# Autodesk Inventor assembly: Inner Channel
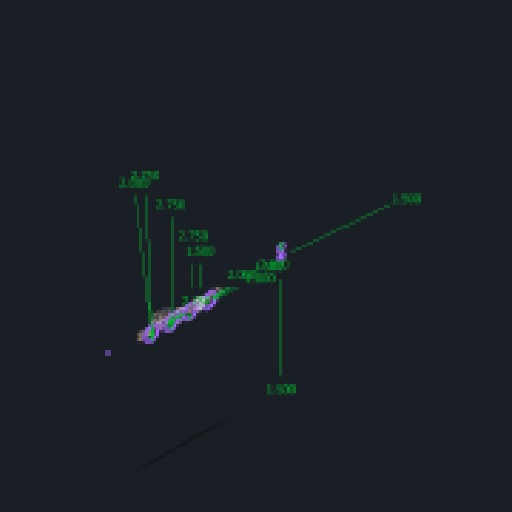
[picture p0: Inventor's stored thumbnail of the model, 512x512]
Saved by Autodesk Inventor 2025.1 (Build 291241000, 241)
## iProperties
Created: 2024-11-04
Part Number: Inner Channel
Document SubType Name: Assembly
Designer: avere
Author: avere
## Documents named in this file (28)
- C:\Users\avere\VEX\High Stakes\CAD\V3\Chassis\Drivebay Right\Inner Channel.iam
- C:\Users\avere\VEX\High Stakes\CAD\V3\Chassis\Drivebay Right\Alu C 1x2x1x30.ipt
- C:\Users\avere\VEX\High Stakes\CAD\V3\Chassis\Drivebay Right\Alu C 1x2x1x6.ipt
- C:\Users\avere\VEX\High Stakes\CAD\V3\Chassis\Drivebay Right\Bearing Flat.ipt
- C:\Users\avere\VEX\High Stakes\CAD\ROBOPROS-CAD-Inventor\Motion\Spacers\Spacer Nylon .500 OD\NSpacer White .500 OD x .250.ipt
- C:\Users\avere\VEX\High Stakes\CAD\ROBOPROS-CAD-Inventor\Motion\Spacers\Spacer Nylon .500 OD.ipt
- C:\Users\avere\VEX\High Stakes\CAD\V3\Chassis\Drivebay Right\Bearing Flat NScrew Slotted Offset.iam
- C:\Users\avere\VEX\High Stakes\CAD\ROBOPROS-CAD-Inventor\Structure\Hardware\Screw Steel - Star\SScrew Star Smooth 1.750.ipt
- C:\Users\avere\VEX\High Stakes\CAD\ROBOPROS-CAD-Inventor\Structure\Hardware\Screw Steel - Star.ipt
- C:\Users\avere\VEX\High Stakes\CAD\ROBOPROS-CAD-Inventor\Structure\Hardware\Screw Steel - Star\SScrew Star Smooth .250.ipt
- C:\Users\avere\VEX\High Stakes\CAD\V3\Chassis\Drivebay Right\Nylon Standoff .875.ipt
- C:\Users\avere\VEX\High Stakes\CAD\ROBOPROS-CAD-Inventor\Motion\Spacers\Spacer Nylon .375 OD\NSpacer .375 OD x .500.ipt
- C:\Users\avere\VEX\High Stakes\CAD\ROBOPROS-CAD-Inventor\Motion\Spacers\Spacer Nylon .375 OD.ipt
- C:\Users\avere\VEX\High Stakes\CAD\ROBOPROS-CAD-Inventor\Structure\Hardware\Nut Nylon\Nut Nylon - White.ipt
- C:\Users\avere\VEX\High Stakes\CAD\ROBOPROS-CAD-Inventor\Structure\Hardware\Nut Nylon.ipt
- C:\Users\avere\VEX\High Stakes\CAD\ROBOPROS-CAD-Inventor\Structure\Hardware\Screw Shoulder Robosource\SScrew Shoulder Smooth 2.000 x .04.ipt
- C:\Users\avere\VEX\High Stakes\CAD\ROBOPROS-CAD-Inventor\Structure\Hardware\Screw Shoulder Robosource.ipt
- C:\Users\avere\VEX\High Stakes\CAD\V3\Chassis\Drivebay Right\Bearing Flat Low Profile 2-Hole.ipt
- C:\Users\avere\VEX\High Stakes\CAD\V3\Chassis\Drivebay Right\1-Post Hex Nut Retainer With Nylon Hardware.iam
- C:\Users\avere\VEX\High Stakes\CAD\V3\Chassis\Drivebay Right\Bearing Flat NScrew Slotted.iam
- C:\Users\avere\VEX\High Stakes\CAD\V3\Chassis\Drivebay Right\Nut Nylon Thread-Forming.ipt
- C:\Users\avere\VEX\High Stakes\CAD\V3\Chassis\Drivebay Right\NScrew Slotted Threaded .500.ipt
- C:\Users\avere\VEX\High Stakes\CAD\V3\Chassis\Drivebay Right\NScrew Pan Head Threaded .250.ipt
- C:\Users\avere\VEX\High Stakes\CAD\ROBOPROS-CAD-Inventor\Structure\Hardware\Screw Shoulder Robosource\SScrew Shoulder Smooth .375 x .12.ipt
- C:\Users\avere\VEX\High Stakes\CAD\ROBOPROS-CAD-Inventor\Motion\Spacers\Spacer Nylon .500 OD\NSpacer White .500 OD x .125.ipt
- C:\Users\avere\VEX\High Stakes\CAD\ROBOPROS-CAD-Inventor\Motion\Spacers\Washer Steel\SWasher .500 OD x .062500\SWasher .500 OD x .062500.ipt
- C:\Users\avere\VEX\High Stakes\CAD\ROBOPROS-CAD-Inventor\Motion\Spacers\Washer Steel\SWasher .500 OD x .062500.ipt
- C:\Users\avere\VEX\High Stakes\CAD\ROBOPROS-CAD-Inventor\Motion\Shaft LS\Bearing Flat.ipt
## Components (56 placed, 20 different names)
1. Alu C 1x2x1x30:1 — Flush:2, Flush:3, Flush:1, Mate:19, Insert:58, Mate:21, Insert:62, Insert:63, Insert:61, Insert:45, Insert:44, Insert:46, Insert:47, Mate:15, Insert:50, Insert:55, Mate:17, Insert:56, Insert:67, Insert:68, Insert:69, Insert:76, Insert:77, Insert:75, Mate:25, Insert:74, Insert:79, Insert:80, Insert:78, Mate:28, Insert:84, Mate:29, Insert:85, Insert:86, Insert:89, Insert:88, Insert:94, Insert:95, Insert:54, Mate:13, Insert:55, Insert:56, Insert:57, Mate:14
2. Alu C 1x2x1x6:1 — Insert:64, Insert:32, Insert:39, Insert:81, Insert:82, Insert:92, Insert:91, Insert:93, Insert:96, Insert:97, Insert:100
3. Bearing Flat:1 — Mate:21, Insert:62, Insert:99
4. Bearing Flat:2 — Insert:63, Insert:20
5. NSpacer White .500 OD x .250:1 — Insert:64, Insert:20
6. SScrew Star Smooth 1.750:1 — Insert:61
7. SScrew Star Smooth .250:2 — Insert:32
8. Nylon Standoff .875:1 — Insert:39
9. NSpacer .375 OD x .500:1 — Insert:54, Insert:51
10. NSpacer .375 OD x .500:2 — Insert:53, Insert:52
11. Nut Nylon - White:1 — Insert:45
12. Nut Nylon - White:2 — Insert:44
13. Nut Nylon - White:3 — Insert:46
14. Nut Nylon - White:4 — Insert:47
15. SScrew Shoulder Smooth 2.000 x .04:1 — Insert:53, Mate:16
16. SScrew Shoulder Smooth 2.000 x .04:2 — Insert:54
17. Bearing Flat Low Profile 2-Hole:1 — Insert:52, Insert:51, Mate:15, Insert:50
18. 1-Post Hex Nut Retainer With Nylon Hardware:1 [sub-assembly] — Mate:16, Insert:55
19. 1-Post Hex Nut Retainer With Nylon Hardware:2 [sub-assembly] — Mate:17, Insert:56
20. NSpacer .375 OD x .500:3 — Insert:73, Insert:70
21. NSpacer .375 OD x .500:4 — Insert:72, Insert:71
22. Nut Nylon - White:5 — Insert:76
23. Nut Nylon - White:6 — Insert:77
24. Nut Nylon - White:7 — Insert:75
25. SScrew Shoulder Smooth 2.000 x .04:3 — Insert:72, Mate:24
26. SScrew Shoulder Smooth 2.000 x .04:4 — Insert:73, Mate:26
27. Bearing Flat Low Profile 2-Hole:2 — Mate:25, Insert:74, Insert:71, Insert:70
28. 1-Post Hex Nut Retainer With Nylon Hardware:3 [sub-assembly] — Insert:79, Mate:24
29. 1-Post Hex Nut Retainer With Nylon Hardware:4 [sub-assembly] — Mate:26, Insert:80
30. Nut Nylon - White:8 — Insert:78
31. Bearing Flat NScrew Slotted:1 [sub-assembly] — Mate:19, Insert:58
32. Nylon Standoff .875:2 — Insert:67
33. Nylon Standoff .875:3 — Insert:68
34. Nylon Standoff .875:4 — Insert:69
35. Nut Nylon Thread-Forming:1 — Insert:81
36. Nut Nylon Thread-Forming:2 — Insert:82
37. Bearing Flat NScrew Slotted Offset:2 [sub-assembly] — Mate:28, Insert:84
38. Bearing Flat Low Profile 2-Hole:3 — Mate:29, Insert:85, Insert:87
39. NScrew Slotted Threaded .500:1 — Insert:86
40. Nut Nylon - White:9 — Insert:87
41. Nut Nylon - White:10 — Insert:89
42. Nut Nylon - White:11 — Insert:88
43. NScrew Pan Head Threaded .250:1 — Insert:92
44. NScrew Pan Head Threaded .250:2 — Insert:91
45. Nylon Standoff .875:5 — Insert:94
46. SScrew Star Smooth .250:3 — Insert:95
47. SScrew Star Smooth 1.750:4 — Insert:93
48. SScrew Shoulder Smooth .375 x .12:5 — Insert:96
49. Nut Nylon Thread-Forming:3 — Insert:97
50. NSpacer White .500 OD x .125:2 — Insert:99, Insert:98
51. SWasher .500 OD x .062500:1 — Insert:100, Insert:98
52. Bearing Flat Low Profile 2-Hole:4 — Insert:54
53. NScrew Slotted Threaded .500:2 — Insert:55
54. Nut Nylon - White:12 — Mate:13
55. Nylon Standoff .875:6 — Insert:56
56. Bearing Flat:3 — Insert:57, Mate:14
## Relationships (71: Insert 56, Mate 13, Flush 2)
- Flush:2 (-38.1 mm): Alu C 1x2x1x30:1
- Flush:3 (-7.9375 mm): Alu C 1x2x1x30:1
- Flush:1 [Mate] (-190.5 mm): Alu C 1x2x1x30:1
- Mate:19: Alu C 1x2x1x30:1 ↔ Bearing Flat NScrew Slotted:1
- Insert:58: Alu C 1x2x1x30:1 ↔ Bearing Flat NScrew Slotted:1
- Mate:21: Alu C 1x2x1x30:1 ↔ Bearing Flat:1
- Insert:62: Alu C 1x2x1x30:1 ↔ Bearing Flat:1
- Insert:63: Alu C 1x2x1x30:1 ↔ Bearing Flat:2
- Insert:64: Alu C 1x2x1x6:1 ↔ NSpacer White .500 OD x .250:1
- Insert:20: Bearing Flat:2 ↔ NSpacer White .500 OD x .250:1
- Insert:61: Alu C 1x2x1x30:1 ↔ SScrew Star Smooth 1.750:1
- Insert:32: Alu C 1x2x1x6:1 ↔ SScrew Star Smooth .250:2
- Insert:39: Alu C 1x2x1x6:1 ↔ Nylon Standoff .875:1
- Insert:45: Alu C 1x2x1x30:1 ↔ Nut Nylon - White:1
- Insert:44: Alu C 1x2x1x30:1 ↔ Nut Nylon - White:2
- Insert:46: Alu C 1x2x1x30:1 ↔ Nut Nylon - White:3
- Insert:47: Alu C 1x2x1x30:1 ↔ Nut Nylon - White:4
- Insert:53 (1.5875 mm): NSpacer .375 OD x .500:2 ↔ SScrew Shoulder Smooth 2.000 x .04:1
- Insert:54 (1.5875 mm): NSpacer .375 OD x .500:1 ↔ SScrew Shoulder Smooth 2.000 x .04:2
- Insert:52 (1.27 mm): NSpacer .375 OD x .500:2 ↔ Bearing Flat Low Profile 2-Hole:1
- Insert:51 (1.27 mm): NSpacer .375 OD x .500:1 ↔ Bearing Flat Low Profile 2-Hole:1
- Mate:15: Alu C 1x2x1x30:1 ↔ Bearing Flat Low Profile 2-Hole:1
- Insert:50: Alu C 1x2x1x30:1 ↔ Bearing Flat Low Profile 2-Hole:1
- Mate:16: SScrew Shoulder Smooth 2.000 x .04:1 ↔ 1-Post Hex Nut Retainer With Nylon Hardware:1
- Insert:55: Alu C 1x2x1x30:1 ↔ 1-Post Hex Nut Retainer With Nylon Hardware:1
- Mate:17: Alu C 1x2x1x30:1 ↔ 1-Post Hex Nut Retainer With Nylon Hardware:2
- Insert:56: Alu C 1x2x1x30:1 ↔ 1-Post Hex Nut Retainer With Nylon Hardware:2
- Insert:67: Alu C 1x2x1x30:1 ↔ Nylon Standoff .875:2
- Insert:68: Alu C 1x2x1x30:1 ↔ Nylon Standoff .875:3
- Insert:69: Alu C 1x2x1x30:1 ↔ Nylon Standoff .875:4
- Insert:76: Alu C 1x2x1x30:1 ↔ Nut Nylon - White:5
- Insert:77: Alu C 1x2x1x30:1 ↔ Nut Nylon - White:6
- Insert:75: Alu C 1x2x1x30:1 ↔ Nut Nylon - White:7
- Insert:72 (1.5875 mm): NSpacer .375 OD x .500:4 ↔ SScrew Shoulder Smooth 2.000 x .04:3
- Insert:73 (1.5875 mm): NSpacer .375 OD x .500:3 ↔ SScrew Shoulder Smooth 2.000 x .04:4
- Mate:25: Alu C 1x2x1x30:1 ↔ Bearing Flat Low Profile 2-Hole:2
- Insert:74: Alu C 1x2x1x30:1 ↔ Bearing Flat Low Profile 2-Hole:2
- Insert:71 (1.27 mm): NSpacer .375 OD x .500:4 ↔ Bearing Flat Low Profile 2-Hole:2
- Insert:70 (1.27 mm): NSpacer .375 OD x .500:3 ↔ Bearing Flat Low Profile 2-Hole:2
- Insert:79: Alu C 1x2x1x30:1 ↔ 1-Post Hex Nut Retainer With Nylon Hardware:3
- Mate:24: SScrew Shoulder Smooth 2.000 x .04:3 ↔ 1-Post Hex Nut Retainer With Nylon Hardware:3
- Mate:26: SScrew Shoulder Smooth 2.000 x .04:4 ↔ 1-Post Hex Nut Retainer With Nylon Hardware:4
- Insert:80: Alu C 1x2x1x30:1 ↔ 1-Post Hex Nut Retainer With Nylon Hardware:4
- Insert:78: Alu C 1x2x1x30:1 ↔ Nut Nylon - White:8
- Insert:81: Alu C 1x2x1x6:1 ↔ Nut Nylon Thread-Forming:1
- Insert:82: Alu C 1x2x1x6:1 ↔ Nut Nylon Thread-Forming:2
- Mate:28: Alu C 1x2x1x30:1 ↔ Bearing Flat NScrew Slotted Offset:2
- Insert:84: Alu C 1x2x1x30:1 ↔ Bearing Flat NScrew Slotted Offset:2
- Mate:29: Alu C 1x2x1x30:1 ↔ Bearing Flat Low Profile 2-Hole:3
- Insert:85: Alu C 1x2x1x30:1 ↔ Bearing Flat Low Profile 2-Hole:3
- Insert:86: Alu C 1x2x1x30:1 ↔ NScrew Slotted Threaded .500:1
- Insert:87 (1.27 mm): Bearing Flat Low Profile 2-Hole:3 ↔ Nut Nylon - White:9
- Insert:89: Alu C 1x2x1x30:1 ↔ Nut Nylon - White:10
- Insert:88: Alu C 1x2x1x30:1 ↔ Nut Nylon - White:11
- Insert:92: Alu C 1x2x1x6:1 ↔ NScrew Pan Head Threaded .250:1
- Insert:91: Alu C 1x2x1x6:1 ↔ NScrew Pan Head Threaded .250:2
- Insert:94: Alu C 1x2x1x30:1 ↔ Nylon Standoff .875:5
- Insert:95: Alu C 1x2x1x30:1 ↔ SScrew Star Smooth .250:3
- Insert:93 (1.5875 mm): Alu C 1x2x1x6:1 ↔ SScrew Star Smooth 1.750:4
- Insert:96: Alu C 1x2x1x6:1 ↔ SScrew Shoulder Smooth .375 x .12:5
- Insert:97 (1.5875 mm): Alu C 1x2x1x6:1 ↔ Nut Nylon Thread-Forming:3
- Insert:99: Bearing Flat:1 ↔ NSpacer White .500 OD x .125:2
- Insert:100 (1.5875 mm): Alu C 1x2x1x6:1 ↔ SWasher .500 OD x .062500:1
- Insert:98: NSpacer White .500 OD x .125:2 ↔ SWasher .500 OD x .062500:1
- [Insert] (1.27 mm): Bearing Flat Low Profile 2-Hole:4 ↔ Nut Nylon - White:12
- Insert:54: Alu C 1x2x1x30:1 ↔ Bearing Flat Low Profile 2-Hole:4
- Mate:13: Alu C 1x2x1x30:1 ↔ Nut Nylon - White:12
- Insert:55: Alu C 1x2x1x30:1 ↔ NScrew Slotted Threaded .500:2
- Insert:56: Alu C 1x2x1x30:1 ↔ Nylon Standoff .875:6
- Insert:57: Alu C 1x2x1x30:1 ↔ Bearing Flat:3
- Mate:14: Alu C 1x2x1x30:1 ↔ Bearing Flat:3
## Named parameters: d78_d53 = 1.27 mm
